# Autodesk Inventor assembly: Servo_Ku_asm
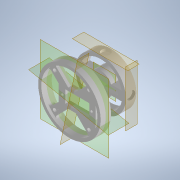
[picture p0: Inventor's stored thumbnail of the model, 180x180]
Saved by Autodesk Inventor 2020 (Build 240168000, 168)
## iProperties
Created: 2022-02-16
Part Number: Servo_Ku_asm
Document SubType Name: Assembly
Designer: sp
Author: sp
## Documents named in this file (3)
- C:\Users\sp\Documents\Rocket\rocket\CAD\Servo_Ku_asm.iam
- C:\Users\sp\Documents\Rocket\rocket\CAD\Servo_Kupplung.ipt
- C:\Users\sp\Documents\Rocket\rocket\CAD\Servo_holder.ipt
## Components (2 placed, 2 different names)
1. Servo_Kupplung:1 — Einfügen:1
2. Servo_holder:1 — Einfügen:1
## Relationships (1: Insert 1)
- Einfügen:1 [Insert] (20 mm): Servo_Kupplung:1 ↔ Servo_holder:1
